# Autodesk Inventor assembly: InjectorBoard2
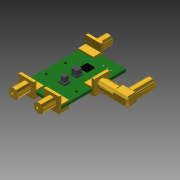
[picture p0: Inventor's stored thumbnail of the model, 180x180]
Saved by Autodesk Inventor 2014 (Build 180170000, 170)
## iProperties
Created: 2015-04-18
Part Number: InjectorBoard2
Document SubType Name: Assembly
Designer: Owner
Author: Owner
## Documents named in this file (8)
- C:\Users\Owner\Documents\APC\FrontEnd\IAM\Common\InjectorBoard2.iam
- C:\Users\Owner\Documents\APC\FrontEnd\IAM\Common\InjectorBoard2.ipt
- C:\Users\Owner\Documents\APC\FrontEnd\IAM\Common\SMA_Edge.ipt
- C:\Users\Owner\Documents\APC\FrontEnd\IAM\Yagi\RFCoupler.ipt
- C:\Users\Owner\Documents\APC\FrontEnd\IAM\Yagi\RFSplitter.ipt
- C:\Users\Owner\Documents\APC\FrontEnd\IAM\Yagi\RFSwitch.ipt
- C:\Users\Owner\Documents\APC\FrontEnd\IAM\Common\3PinHeader.ipt
- C:\Users\Owner\Documents\APC\FrontEnd\IAM\Common\SMA_RightAngle.ipt
## Components (10 placed, 7 different names)
1. InjectorBoard2:1 — Mate:9, Mate:10, Mate:11, Flush:5, Flush:6, Flush:7, Flush:8, Flush:9, Flush:10, Mate:12, Flush:11, Flush:12, Mate:13, Mate:14, Mate:15, Mate:16, Mate:17, Mate:18, Mate:19, Mate:20, Flush:13, Flush:14, Flush:15, Flush:16, Angle:1
2. RFCoupler:1 — Mate:10, Flush:7, Flush:8
3. RFSplitter:1 — Mate:9, Flush:9, Flush:10
4. RFSwitch:1 — Mate:11, Flush:5, Flush:6
5. 3PinHeader:1 — Mate:12, Flush:11, Flush:12
6. SMA_Edge:1 — Mate:16, Mate:18, Flush:16
7. SMA_Edge:2 — Mate:15, Mate:17, Flush:15
8. SMA_Edge:3 — Mate:13, Mate:19, Flush:13
9. SMA_Edge:4 — Mate:14, Mate:20, Flush:14, Mate:21, Mate:22
10. SMA_RightAngle:1 — Mate:21, Mate:22, Angle:1
## Relationships (27: Mate 14, Flush 12, Angle 1)
- Mate:9: InjectorBoard2:1 ↔ RFSplitter:1
- Mate:10: InjectorBoard2:1 ↔ RFCoupler:1
- Mate:11: InjectorBoard2:1 ↔ RFSwitch:1
- Flush:5 (10.16 mm): InjectorBoard2:1 ↔ RFSwitch:1
- Flush:6 (9.7536 mm): InjectorBoard2:1 ↔ RFSwitch:1
- Flush:7 (10.2616 mm): InjectorBoard2:1 ↔ RFCoupler:1
- Flush:8 (16.9164 mm): InjectorBoard2:1 ↔ RFCoupler:1
- Flush:9 (9.779 mm): InjectorBoard2:1 ↔ RFSplitter:1
- Flush:10 (24.9682 mm): InjectorBoard2:1 ↔ RFSplitter:1
- Mate:12: InjectorBoard2:1 ↔ 3PinHeader:1
- Flush:11 (4.1148 mm): InjectorBoard2:1 ↔ 3PinHeader:1
- Flush:12 (2.4384 mm): InjectorBoard2:1 ↔ 3PinHeader:1
- Mate:13: InjectorBoard2:1 ↔ SMA_Edge:3
- Mate:14: InjectorBoard2:1 ↔ SMA_Edge:4
- Mate:15: InjectorBoard2:1 ↔ SMA_Edge:2
- Mate:16: InjectorBoard2:1 ↔ SMA_Edge:1
- Mate:17: InjectorBoard2:1 ↔ SMA_Edge:2
- Mate:18: InjectorBoard2:1 ↔ SMA_Edge:1
- Mate:19: InjectorBoard2:1 ↔ SMA_Edge:3
- Mate:20: InjectorBoard2:1 ↔ SMA_Edge:4
- Flush:13: InjectorBoard2:1 ↔ SMA_Edge:3
- Flush:14 (12.0142 mm): InjectorBoard2:1 ↔ SMA_Edge:4
- Flush:15: InjectorBoard2:1 ↔ SMA_Edge:2
- Flush:16: InjectorBoard2:1 ↔ SMA_Edge:1
- Mate:21: SMA_Edge:4 ↔ SMA_RightAngle:1
- Mate:22 (2 mm): SMA_Edge:4 ↔ SMA_RightAngle:1
- Angle:1 (0 deg): InjectorBoard2:1 ↔ SMA_RightAngle:1
